# Autodesk Inventor assembly: Wheel-Axel Assembly
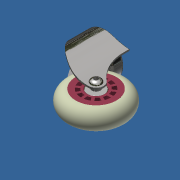
[picture p0: Inventor's stored thumbnail of the model, 180x180]
Saved by Autodesk Inventor 2018 (Build 220112000, 112)
## iProperties
Created: 2018-03-27
Part Number: Wheel-Axel Assembly
Document SubType Name: Assembly
Designer: Cole
Author: Cole
## Documents named in this file (6)
- D:\Cole\Documents\GitHub\SchoolCAD\ReverseEngineering\Wheel-Axel Assembly.iam
- D:\Cole\Documents\GitHub\SchoolCAD\ReverseEngineering\Axel-Male.ipt
- D:\Cole\Documents\GitHub\SchoolCAD\ReverseEngineering\Axel-Female.ipt
- D:\Cole\Documents\GitHub\SchoolCAD\ReverseEngineering\Axel Buffer.ipt
- D:\Cole\Documents\GitHub\SchoolCAD\ReverseEngineering\Axel Mount.ipt
- D:\Cole\Documents\GitHub\SchoolCAD\ReverseEngineering\Wheel.ipt
## Components (6 placed, 5 different names)
1. Axel-Male:1 — Insert:1
2. Axel-Female:1 — Insert:1, Insert:2, Insert:5
3. Axel Buffer:1 — Insert:4
4. Axel Buffer:2 — Insert:3
5. Axel Mount:1 — Insert:2, Insert:3, Insert:4
6. Wheel:1 — Insert:5
## Relationships (5: Insert 5)
- Insert:1: Axel-Male:1 ↔ Axel-Female:1
- Insert:2: Axel-Female:1 ↔ Axel Mount:1
- Insert:3: Axel Buffer:2 ↔ Axel Mount:1
- Insert:4: Axel Buffer:1 ↔ Axel Mount:1
- Insert:5 (0.9779 mm): Axel-Female:1 ↔ Wheel:1
